# Autodesk Inventor assembly: head_right
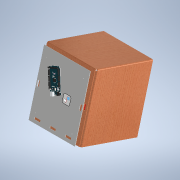
[picture p0: Inventor's stored thumbnail of the model, 180x180]
Saved by Autodesk Inventor 2021.1 (Build 251245010, 245A)
## iProperties
Created: 2023-01-13
Part Number: head_right
Document SubType Name: Assembly
Designer: zmoze
Author: zmoze
## Documents named in this file (7)
- C:\Users\zmoze\OneDrive\Рабочий стол\GrabCAD\Smile_2022-2023\head_right.iam
- C:\Users\zmoze\OneDrive\Рабочий стол\GrabCAD\Smile_2022-2023\face_right.ipt
- C:\Users\zmoze\OneDrive\Рабочий стол\GrabCAD\Smile_2022-2023\head_without_face_right.ipt
- C:\Users\zmoze\OneDrive\Рабочий стол\GrabCAD\Smile_2022-2023\панель_с_электроникой.ipt
- C:\Users\zmoze\OneDrive\Рабочий стол\GrabCAD\Smile_2022-2023\arduino_MEGA2560.iam
- C:\Users\zmoze\OneDrive\Рабочий стол\GrabCAD\Smile_2022-2023\рот.ipt
- C:\Users\zmoze\OneDrive\Рабочий стол\GrabCAD\Smile_2022-2023\глаз.ipt
## Components (7 placed, 6 different names)
1. face_right:1 — Совмещение:1, Совмещение:2, Совмещение:3, Заподлицо:1, Заподлицо:3, Заподлицо:4, Заподлицо:5, Совмещение:7, Совмещение:8, Заподлицо:6, Заподлицо:7, Совмещение:9, Совмещение:10
2. head_without_face_right:1 — Совмещение:1, Совмещение:2, Совмещение:3, Заподлицо:1, Заподлицо:2, Совмещение:4, Совмещение:5
3. панель_с_электроникой:1 — Заподлицо:2, Совмещение:4, Совмещение:5, Совмещение:6
4. arduino_MEGA2560:1 [sub-assembly] — Совмещение:6
5. рот:1 — Заподлицо:5, Совмещение:9, Совмещение:10
6. глаз:1 — Заподлицо:4, Совмещение:7, Заподлицо:7
7. глаз:2 — Заподлицо:3, Совмещение:8, Заподлицо:6
## Relationships (17: Mate 10, Flush 7)
- Совмещение:1 [Mate]: face_right:1 ↔ head_without_face_right:1
- Совмещение:2 [Mate]: face_right:1 ↔ head_without_face_right:1
- Совмещение:3 [Mate]: face_right:1 ↔ head_without_face_right:1
- Заподлицо:1 [Flush]: face_right:1 ↔ head_without_face_right:1
- Заподлицо:2 [Flush] (-11 mm): head_without_face_right:1 ↔ панель_с_электроникой:1
- Совмещение:4 [Mate]: head_without_face_right:1 ↔ панель_с_электроникой:1
- Совмещение:5 [Mate] (15 mm): head_without_face_right:1 ↔ панель_с_электроникой:1
- Совмещение:6 [Mate] (10 mm): панель_с_электроникой:1 ↔ arduino_MEGA2560:1
- Заподлицо:3 [Flush]: face_right:1 ↔ глаз:2
- Заподлицо:4 [Flush]: face_right:1 ↔ глаз:1
- Заподлицо:5 [Flush]: face_right:1 ↔ рот:1
- Совмещение:7 [Mate] (30 mm): face_right:1 ↔ глаз:1
- Совмещение:8 [Mate] (30 mm): face_right:1 ↔ глаз:2
- Заподлицо:6 [Flush] (-30 mm): face_right:1 ↔ глаз:2
- Заподлицо:7 [Flush] (-30 mm): face_right:1 ↔ глаз:1
- Совмещение:9 [Mate] (37.75 mm): face_right:1 ↔ рот:1
- Совмещение:10 [Mate] (20 mm): face_right:1 ↔ рот:1
